# Autodesk Inventor assembly: robot
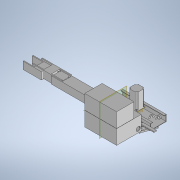
[picture p0: Inventor's stored thumbnail of the model, 180x180]
Saved by Autodesk Inventor 2020 (Build 240168000, 168)
## iProperties
Created: 2021-03-19
Part Number: robot
Document SubType Name: Assembly
Designer: super
Author: super
## Documents named in this file (14)
- C:\desk\promissionsave\inventor\robot\robot morango.iam
- C:\desk\promissionsave\inventor\robot\corpo.ipt
- C:\desk\promissionsave\inventor\robot\servospt70.ipt
- C:\desk\promissionsave\inventor\robot\balde.ipt
- C:\desk\promissionsave\inventor\robot\armj1.ipt
- C:\desk\promissionsave\inventor\robot\armj2.ipt
- C:\desk\promissionsave\inventor\robot\nema23.ipt
- C:\desk\promissionsave\inventor\robot\armj3.ipt
- C:\desk\promissionsave\inventor\robot\armj4.ipt
- C:\desk\promissionsave\inventor\robot\guia.ipt
- C:\desk\promissionsave\inventor\container\c150x43x15x200.ipt
- C:\desk\promissionsave\inventor\robot\gira.ipt
- C:\desk\promissionsave\inventor\robot\guia_MIR.ipt
- C:\desk\promissionsave\inventor\robot\guia_MIR_MIR.ipt
## Components (20 placed, 13 different names)
1. corpo:1 — Mate:5, Flush:2, Mate:7, Flush:4, Flush:5, Mate:8, Mate:9, Flush:6, Mate:15, Mate:17, Mate:18, Flush:11, Symmetry:1, Mate:22
2. servospt70:1 — Mate:8, Mate:9, Flush:6, Rotational:1
3. balde:1 — Mate:7, Flush:4, Flush:5, Symmetry:1
4. servospt70:2 — Mate:10, Mate:11, Flush:7
5. armj1:1 — Rotational:1, Mate:10, Mate:11, Flush:7, Mate:12, Flush:8, Mate:14, Flush:9
6. armj1:2 — Mate:12, Mate:13, Flush:8
7. armj1:3 — Mate:13
8. armj2:1 — Mate:14, Flush:9, Mate:15, Mate:16, Flush:10
9. armj3:1 — Mate:16, Flush:10, Mate:19
10. servospt70:3
11. armj4:1 — Mate:19
12. guia:3
13. guia:4 — Flush:13
14. c150x43x15x200:1 — Mate:20, Flush:12, Flush:14, Flush:15, Tangent:1
15. guia:7
16. guia:9 — Tangent:1
17. gira:1 — Flush:12, Flush:13, Mate:21, Mate:22
18. guia_MIR:1
19. guia_MIR_MIR:1
20. nema23:1 — Mate:17, Mate:18, Flush:11
## Relationships (33: Mate 17, Flush 13, RevoluteJoint 1, Tangent 1, Symmetry 1)
- Mate:5: corpo:1
- Flush:2: corpo:1
- Mate:7 (1 mm): corpo:1 ↔ balde:1
- Flush:4: corpo:1 ↔ balde:1
- Flush:5: corpo:1 ↔ balde:1
- Mate:8: corpo:1 ↔ servospt70:1
- Mate:9: corpo:1 ↔ servospt70:1
- Flush:6: corpo:1 ↔ servospt70:1
- Rotational:1 [RevoluteJoint]: servospt70:1 ↔ armj1:1
- Mate:10: servospt70:2 ↔ armj1:1
- Mate:11: servospt70:2 ↔ armj1:1
- Flush:7 (10 mm): servospt70:2 ↔ armj1:1
- Mate:12: armj1:1 ↔ armj1:2
- Mate:13: armj1:2 ↔ armj1:3
- Flush:8: armj1:1 ↔ armj1:2
- Mate:14: armj1:1 ↔ armj2:1
- Flush:9: armj1:1 ↔ armj2:1
- Mate:15 (40 mm): corpo:1 ↔ armj2:1
- Mate:16: armj2:1 ↔ armj3:1
- Flush:10: armj2:1 ↔ armj3:1
- Mate:17 (-50 mm): corpo:1 ↔ nema23:1
- Mate:18 (50 mm): corpo:1 ↔ nema23:1
- Flush:11 (81.5 mm): corpo:1 ↔ nema23:1
- Mate:19: armj3:1 ↔ armj4:1
- Mate:20 (-50 mm): c150x43x15x200:1
- Flush:12: c150x43x15x200:1 ↔ gira:1
- Flush:13: guia:4 ↔ gira:1
- Flush:14 (-1.5 mm): c150x43x15x200:1
- Flush:15 (-150 mm): c150x43x15x200:1
- Tangent:1: c150x43x15x200:1 ↔ guia:9
- Symmetry:1: corpo:1 ↔ balde:1
- Mate:21: gira:1
- Mate:22 (10 mm): corpo:1 ↔ gira:1
